# Autodesk Inventor assembly: 4x2
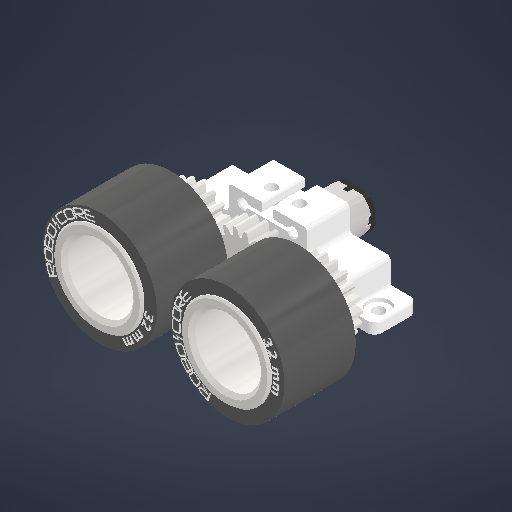
[picture p0: Inventor's stored thumbnail of the model, 512x512]
Saved by Autodesk Inventor 2026.1 (Build 301233020, 233B)
## iProperties
Created: 2026-02-10
Part Number: 4x2
Document SubType Name: Assembly
Designer: celio
Author: celio
## Documents named in this file (7)
- C:\Users\celio\OneDrive\Documentos\Inventor\ZeGuia\Montagem\4x2\Base\4x2.iam
- C:\Users\celio\OneDrive\Documentos\Inventor\ZeGuia\Motores\N20\N20 DC MOTOR.ipt
- C:\Users\celio\OneDrive\Documentos\Inventor\ZeGuia\Montagem\4x2\Suporte.ipt
- C:\Users\celio\OneDrive\Documentos\Inventor\ZeGuia\Montagem\4x2\Parafuso m3x30.ipt
- C:\Users\celio\OneDrive\Documentos\Inventor\ZeGuia\Montagem\4x2\Engrenagem motor 20 dentes.ipt
- C:\Users\celio\OneDrive\Documentos\Inventor\ZeGuia\Montagem\4x2\Engrenagem rodas 20 dentes.ipt
- C:\Users\celio\OneDrive\Documentos\Inventor\ZeGuia\Roda\parts\StickyMAX-32mm-Pneu-Loja_Predeterminada.ipt
## Components (9 placed, 5 different names)
1. N20 DC MOTOR:1 — Coincidente:1, Coincidente:3, Alinhado:4, Coincidente:4, Alinhado:5, Coincidente:10
2. Suporte:1 — Alinhado:4, Coincidente:4, Alinhado:5, Rígida:2, Rígida:3, Coincidente:5, Coincidente:6, Coincidente:9
3. Parafuso m3x30:1 — Rígida:2, Coincidente:7
4. Parafuso m3x30:2 — Rígida:3, Coincidente:8
5. Engrenagem reta1:1 — Coincidente:9, Coincidente:10, Rotação:1, Rotação:2
6. Engrenagem reta1:2 — Rígida:5, Coincidente:6, Coincidente:8, Rotação:2
7. Engrenagem reta1:3 — Rígida:4, Coincidente:5, Coincidente:7, Rotação:1
8. StickyMAX-32mm-Pneu-Loja_Predeterminada:1 — Rígida:5
9. StickyMAX-32mm-Pneu-Loja_Predeterminada:2 — Rígida:4
## Relationships (22: Mate 9, WeldJoint 4, Angle 3, Symmetry 2, Flush 2, RelateRotation 2)
- Ângulo:1 [Angle] (0 deg)
- Simetria:1 [Symmetry]
- Coincidente:1 [Mate] (-5 mm): N20 DC MOTOR:1
- Ângulo:2 [Angle] (0 deg)
- Ângulo:3 [Angle] (0 deg)
- Simetria:2 [Symmetry]
- Coincidente:3 [Mate] (-6 mm): N20 DC MOTOR:1
- Alinhado:4 [Flush]: N20 DC MOTOR:1 ↔ Suporte:1
- Coincidente:4 [Mate]: N20 DC MOTOR:1 ↔ Suporte:1
- Alinhado:5 [Flush]: N20 DC MOTOR:1 ↔ Suporte:1
- Rígida:2 [WeldJoint]: Suporte:1 ↔ Parafuso m3x30:1
- Rígida:3 [WeldJoint]: Suporte:1 ↔ Parafuso m3x30:2
- Rígida:4 [WeldJoint]: Engrenagem reta1:3 ↔ StickyMAX-32mm-Pneu-Loja_Predeterminada:2
- Rígida:5 [WeldJoint]: Engrenagem reta1:2 ↔ StickyMAX-32mm-Pneu-Loja_Predeterminada:1
- Coincidente:5 [Mate] (1 mm): Suporte:1 ↔ Engrenagem reta1:3
- Coincidente:6 [Mate] (1 mm): Suporte:1 ↔ Engrenagem reta1:2
- Coincidente:7 [Mate]: Parafuso m3x30:1 ↔ Engrenagem reta1:3
- Coincidente:8 [Mate]: Parafuso m3x30:2 ↔ Engrenagem reta1:2
- Coincidente:9 [Mate] (1.5 mm): Suporte:1 ↔ Engrenagem reta1:1
- Coincidente:10 [Mate]: N20 DC MOTOR:1 ↔ Engrenagem reta1:1
- Rotação:1 [RelateRotation] (1 ul): Engrenagem reta1:1 ↔ Engrenagem reta1:3
- Rotação:2 [RelateRotation] (1 ul): Engrenagem reta1:1 ↔ Engrenagem reta1:2
